# Autodesk Inventor assembly: Assembly1
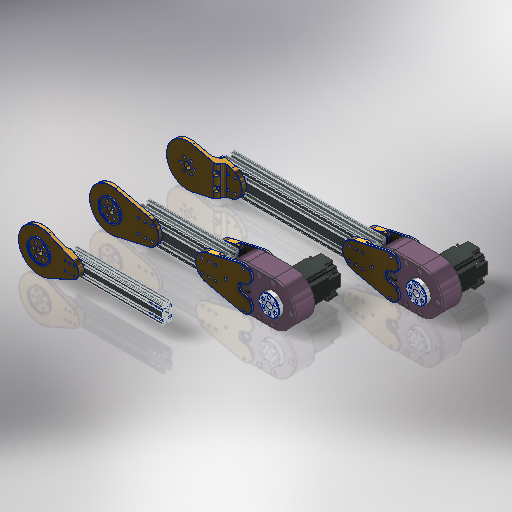
[picture p0: Inventor's stored thumbnail of the model, 512x512]
Saved by Autodesk Inventor 2026 (Build 300175000, 175)
## iProperties
Created: 2025-12-02
Part Number: Assembly1
Document SubType Name: Assembly
Designer: DanielFGarzon
Author: DanielFGarzon
## Documents named in this file (4)
- D:\POLIMI\3RD SEMESTER\Industrial Robotics\Project\Mine\Assembly1.iam
- D:\POLIMI\3RD SEMESTER\Industrial Robotics\Project\Mine\Link_01_Assembly_V02.iam
- D:\POLIMI\3RD SEMESTER\Industrial Robotics\Project\Mine\Link_02_Assembly_V02.iam
- D:\POLIMI\3RD SEMESTER\Industrial Robotics\Project\Mine\Link_03_Assembly_V02.iam
## Components (3 placed, 3 different names)
1. Link_01_Assembly_V02:1 [sub-assembly] — Flush:1, Mate:1
2. Link_02_Assembly_V02:1 [sub-assembly] — Flush:1, Mate:1, Mate:2
3. Link_03_Assembly_V02:1 [sub-assembly] — Mate:2
## Relationships (3: Mate 2, Flush 1)
- Flush:1: Link_01_Assembly_V02:1 ↔ Link_02_Assembly_V02:1
- Mate:1: Link_01_Assembly_V02:1 ↔ Link_02_Assembly_V02:1
- Mate:2: Link_02_Assembly_V02:1 ↔ Link_03_Assembly_V02:1
